# Autodesk Inventor assembly: BoardAssy
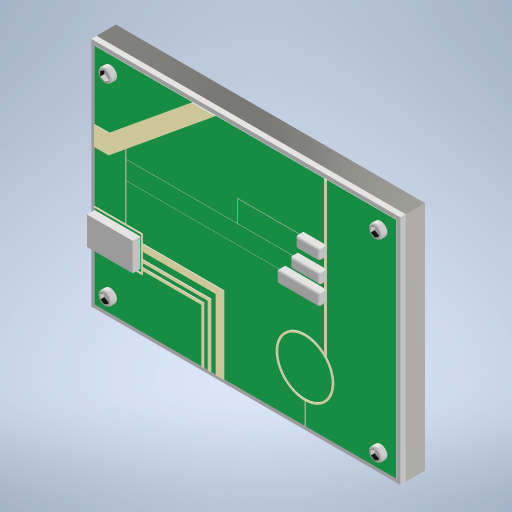
[picture p0: Inventor's stored thumbnail of the model, 512x512]
Saved by Autodesk Inventor 2023 (Build 270158000, 158)
## iProperties
Created: 2022-11-08
Part Number: BoardAssy
Document SubType Name: Assembly
Designer: 223076749
Author: 223076749
## Documents named in this file (4)
- C:\Users\223076749\Documents\BoardAssy.iam
- C:\Users\223076749\Documents\Base Plate.ipt
- C:\Users\223076749\Documents\Board.ipt
- C:\Users\223076749\Documents\Bolt.ipt
## Components (6 placed, 3 different names)
1. Base Plate:1 — Mate:1, Flush:1, Flush:2
2. Board:1 — Mate:1, Flush:1, Flush:2, Cylindrical:1, Cylindrical:2, Cylindrical:3, Cylindrical:4, Mate:2, Mate:3, Mate:4, Mate:5
3. Bolt:1 — Cylindrical:2, Mate:3
4. Bolt:2 — Cylindrical:4, Mate:2
5. Bolt:3 — Cylindrical:1, Mate:4
6. Bolt:4 — Cylindrical:3, Mate:5
## Relationships (11: Mate 5, CylindricalJoint 4, Flush 2)
- Mate:1: Base Plate:1 ↔ Board:1
- Flush:1: Base Plate:1 ↔ Board:1
- Flush:2: Base Plate:1 ↔ Board:1
- Cylindrical:1: Board:1 ↔ Bolt:3
- Cylindrical:2: Board:1 ↔ Bolt:1
- Cylindrical:3: Board:1 ↔ Bolt:4
- Cylindrical:4: Board:1 ↔ Bolt:2
- Mate:2: Board:1 ↔ Bolt:2
- Mate:3: Board:1 ↔ Bolt:1
- Mate:4: Board:1 ↔ Bolt:3
- Mate:5: Board:1 ↔ Bolt:4
